# Autodesk Inventor assembly: DraftAssembly
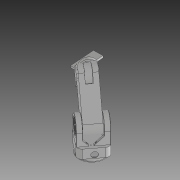
[picture p0: Inventor's stored thumbnail of the model, 180x180]
Saved by Autodesk Inventor 2020 (Build 240168000, 168)
## iProperties
Created: 2021-03-19
Part Number: DraftAssembly
Document SubType Name: Assembly
Designer: DDeGo
Author: DDeGo
## Documents named in this file (15)
- C:\Users\DDeGo\Documents\Drew\Projects\OS-ARM\cad\FirstDraft\DraftAssembly.iam
- C:\Users\DDeGo\Documents\Drew\Projects\OS-ARM\cad\FirstDraft\Base.ipt
- C:\Users\DDeGo\Documents\Drew\Projects\OS-ARM\cad\FirstDraft\Link1.ipt
- C:\Users\DDeGo\Documents\Drew\Projects\OS-ARM\cad\FirstDraft\Link2.ipt
- C:\Users\DDeGo\Documents\Drew\Projects\OS-ARM\cad\FirstDraft\CamBracket.ipt
- C:\Users\DDeGo\Documents\Drew\Projects\OS-ARM\cad\FirstDraft\Wrist.ipt
- C:\Users\DDeGo\Documents\Drew\Projects\OS-ARM\cad\FirstDraft\J1_Base.ipt
- C:\Users\DDeGo\Documents\Drew\Projects\OS-ARM\cad\FirstDraft\J1_Drive.iam
- C:\Users\DDeGo\Documents\Drew\Projects\OS-ARM\cad\FirstDraft\Link3.ipt
- C:\Users\DDeGo\Documents\Drew\Projects\OS-ARM\cad\OTS\Nema 17 22mm.ipt
- C:\Users\DDeGo\Documents\Drew\Projects\OS-ARM\cad\OTS\NEMA 23 - 41mm.ipt
- C:\Users\DDeGo\Documents\Drew\Projects\OS-ARM\cad\HarmonicDrive75mm\HarmonicDrive75mm.iam
- C:\Users\DDeGo\Documents\Drew\Projects\OS-ARM\cad\OTS\6815 bearing.ipt
- C:\Users\DDeGo\Documents\Drew\Projects\OS-ARM\cad\FirstDraft\J1_idlebracket.ipt
- C:\Users\DDeGo\Documents\Drew\Projects\OS-ARM\cad\FirstDraft\fakepully.ipt
## Components (17 placed, 14 different names)
1. Base:1 — Mate:42, Mate:43
2. Link1:1 — Mate:19, Mate:30, Mate:33, Mate:34, Mate:35, Mate:40, Mate:41, Mate:46, Mate:49, Mate:52, Mate:53
3. Link2:1 — Mate:23, Mate:24, Mate:36, Mate:37, Mate:38
4. CamBracket:1 — Mate:9, Mate:12
5. Wrist:1 — Mate:9, Mate:12, Mate:25, Mate:26, Mate:27
6. J1_Base:1 — Mate:14, Angle:1, Mate:42, Mate:43, Mate:44, Flush:2, Mate:45, Flush:4, Mate:47, Mate:48, Mate:50, Mate:51, Angle:2
7. J1_Drive:1 [sub-assembly] — Mate:14, Mate:19, Angle:1, Mate:40, Mate:41, Mate:44, Flush:2
8. Link3:1 — Mate:23, Mate:24, Mate:25, Mate:26, Flush:1, Angle:2
9. Nema 17 22mm:1 — Flush:1, Mate:27
10. NEMA 23 - 41mm:1 — Mate:30, Mate:49
11. HarmonicDrive75mm:1 [sub-assembly] — Mate:31, Mate:32, Mate:35, Mate:36, Mate:37, Mate:38
12. 6815 bearing:1 — Mate:31, Mate:32, Mate:33, Mate:34
13. Nema 17 22mm:2
14. NEMA 23 - 41mm:2 — Mate:47, Mate:48
15. J1_idlebracket:1 — Mate:45, Flush:4, Mate:46
16. NEMA 23 - 41mm:3 — Mate:50, Mate:51
17. fakepully:1 — Mate:52, Mate:53
## Relationships (37: Mate 32, Flush 3, Angle 2)
- Mate:9: CamBracket:1 ↔ Wrist:1
- Mate:12: CamBracket:1 ↔ Wrist:1
- Mate:14: J1_Base:1 ↔ J1_Drive:1
- Mate:19: Link1:1 ↔ J1_Drive:1
- Mate:23: Link2:1 ↔ Link3:1
- Mate:24: Link2:1 ↔ Link3:1
- Mate:25: Wrist:1 ↔ Link3:1
- Mate:26: Wrist:1 ↔ Link3:1
- Flush:1: Link3:1 ↔ Nema 17 22mm:1
- Mate:27: Wrist:1 ↔ Nema 17 22mm:1
- Mate:30 (5 mm): Link1:1 ↔ NEMA 23 - 41mm:1
- Angle:1 (0 deg): J1_Base:1 ↔ J1_Drive:1
- Mate:31: HarmonicDrive75mm:1 ↔ 6815 bearing:1
- Mate:32: HarmonicDrive75mm:1 ↔ 6815 bearing:1
- Mate:33: Link1:1 ↔ 6815 bearing:1
- Mate:34: Link1:1 ↔ 6815 bearing:1
- Mate:35: Link1:1 ↔ HarmonicDrive75mm:1
- Mate:36: Link2:1 ↔ HarmonicDrive75mm:1
- Mate:37: Link2:1 ↔ HarmonicDrive75mm:1
- Mate:38: Link2:1 ↔ HarmonicDrive75mm:1
- Mate:40: Link1:1 ↔ J1_Drive:1
- Mate:41: Link1:1 ↔ J1_Drive:1
- Mate:42: Base:1 ↔ J1_Base:1
- Mate:43: Base:1 ↔ J1_Base:1
- Mate:44: J1_Base:1 ↔ J1_Drive:1
- Flush:2: J1_Base:1 ↔ J1_Drive:1
- Mate:45: J1_Base:1 ↔ J1_idlebracket:1
- Flush:4: J1_Base:1 ↔ J1_idlebracket:1
- Mate:46: Link1:1 ↔ J1_idlebracket:1
- Mate:47: J1_Base:1 ↔ NEMA 23 - 41mm:2
- Mate:48 (25 mm): J1_Base:1 ↔ NEMA 23 - 41mm:2
- Mate:49: Link1:1 ↔ NEMA 23 - 41mm:1
- Mate:50: J1_Base:1 ↔ NEMA 23 - 41mm:3
- Mate:51: J1_Base:1 ↔ NEMA 23 - 41mm:3
- Mate:52: Link1:1 ↔ fakepully:1
- Mate:53: Link1:1 ↔ fakepully:1
- Angle:2 (0 deg): J1_Base:1 ↔ Link3:1
